# Autodesk Inventor assembly: Robot
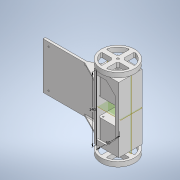
[picture p0: Inventor's stored thumbnail of the model, 180x180]
Saved by Autodesk Inventor 2021 (Build 250183000, 183)
## iProperties
Created: 2021-03-14
Part Number: Robot
Document SubType Name: Assembly
Designer: awitc
Author: awitc
## Documents named in this file (5)
- C:\Users\awitc\Documents\Designed Parts\selfBalancingRobot\Robot.iam
- C:\Users\awitc\Documents\Designed Parts\selfBalancingRobot\stepperMotor.ipt
- C:\Users\awitc\Documents\Designed Parts\selfBalancingRobot\stepperMotorLink.ipt
- C:\Users\awitc\Documents\Designed Parts\selfBalancingRobot\support.ipt
- C:\Users\awitc\Documents\Designed Parts\selfBalancingRobot\wheel.ipt
## Components (6 placed, 4 different names)
1. stepperMotorLink:1 — Insert:7, Insert:8, Insert:9, Insert:10, Mate:1, Flush:1, Flush:2, Insert:11, Insert:12
2. stepperMotor:2 — Insert:7, Insert:8
3. support:1 — Mate:1, Flush:1, Flush:2
4. stepperMotor:3 — Insert:9, Insert:10
5. wheel:1 — Insert:12
6. wheel:2 — Insert:11
## Relationships (9: Insert 6, Flush 2, Mate 1)
- Insert:7: stepperMotorLink:1 ↔ stepperMotor:2
- Insert:8: stepperMotorLink:1 ↔ stepperMotor:2
- Insert:9: stepperMotorLink:1 ↔ stepperMotor:3
- Insert:10: stepperMotorLink:1 ↔ stepperMotor:3
- Mate:1: stepperMotorLink:1 ↔ support:1
- Flush:1: stepperMotorLink:1 ↔ support:1
- Flush:2: stepperMotorLink:1 ↔ support:1
- Insert:11: stepperMotorLink:1 ↔ wheel:2
- Insert:12: stepperMotorLink:1 ↔ wheel:1
